# Autodesk Inventor assembly: 組合1
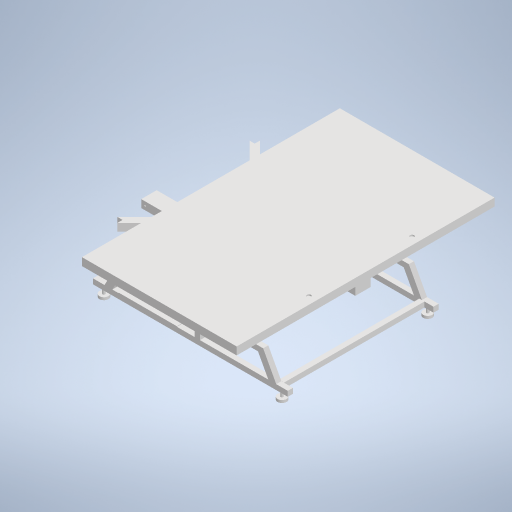
[picture p0: Inventor's stored thumbnail of the model, 512x512]
Saved by Autodesk Inventor 2024 (Build 280153000, 153)
## iProperties
Created: 2024-10-15
Part Number: 組合1
Document SubType Name: Assembly
Designer: jerry
Author: jerry
## Documents named in this file (21)
- C:\HeadTurner\HeadTurner\Linear Actuator\CAD Models\Inventor Model\組合1.iam
- C:\HeadTurner\HeadTurner\Linear Actuator\CAD Models\Inventor Model\Body Actuator.ipt
- C:\HeadTurner\HeadTurner\Linear Actuator\CAD Models\Inventor Model\DOF1.ipt
- C:\HeadTurner\HeadTurner\Linear Actuator\CAD Models\Inventor Model\DOF2.ipt
- C:\HeadTurner\HeadTurner\Linear Actuator\CAD Models\Inventor Model\DOF3.ipt
- C:\HeadTurner\HeadTurner\Linear Actuator\CAD Models\Inventor Model\DOF4.ipt
- C:\HeadTurner\HeadTurner\Linear Actuator\CAD Models\Inventor Model\DOF5.ipt
- C:\HeadTurner\HeadTurner\Linear Actuator\CAD Models\Inventor Model\DOF6.ipt
- C:\HeadTurner\HeadTurner\Linear Actuator\CAD Models\Inventor Model\DOF7.ipt
- C:\HeadTurner\HeadTurner\Linear Actuator\CAD Models\Inventor Model\DOF8.ipt
- C:\HeadTurner\HeadTurner\Linear Actuator\CAD Models\Inventor Model\DOF9.ipt
- C:\HeadTurner\HeadTurner\Linear Actuator\CAD Models\Inventor Model\DOF10.ipt
- C:\Users\jerry\OneDrive\Documents\Mattress.ipt
- C:\Users\jerry\OneDrive\Documents\Mattress2.ipt
- C:\Users\jerry\OneDrive\Documents\DOF11.ipt
- C:\Users\jerry\OneDrive\Documents\MotorPart1.ipt
- C:\Users\jerry\OneDrive\Documents\MotorPart2.ipt
- C:\Users\jerry\OneDrive\Documents\MotorPart3.ipt
- C:\Users\jerry\OneDrive\Documents\Cranker1.ipt
- C:\Users\jerry\OneDrive\Documents\MotorPart3_MIR.ipt
- C:\Users\jerry\OneDrive\Documents\Cranker1_MIR.ipt
## Components (22 placed, 20 different names)
1. Body Actuator:1 — 齊平:1, 齊平:3, 齊平:11
2. DOF1:1 — 齊平:1, 齊平:2
3. DOF2:1 — 齊平:2, 齊平:4, 齊平:6
4. DOF3:1 — 齊平:3
5. DOF4:1 — 齊平:4, 齊平:5
6. DOF5:1 — 齊平:5, 齊平:7, 齊平:8
7. DOF6:1 — 齊平:6, 齊平:13, 貼合:1, 貼合:2
8. DOF7:1 — 齊平:7, 齊平:10
9. DOF8:1 — 齊平:8, 齊平:9
10. DOF9:1 — 齊平:9
11. DOF10:1 — 齊平:10, 齊平:14, 貼合:3, 貼合:4
12. Mattress:1 — 齊平:11, 齊平:12
13. Mattress2:1 — 齊平:12
14. DOF11:1 — 齊平:13, 貼合:1, 貼合:2
15. MotorPart1:1 — 齊平:14, 貼合:3, 插入:1, 貼合:5
16. MotorPart1:2 — 貼合:4, 齊平:15, 齊平:16
17. MotorPart2:1 — 齊平:15
18. MotorPart2:2 — 插入:1
19. MotorPart3:1 — 齊平:16, 齊平:17
20. Cranker1:1 — 齊平:17
21. MotorPart3_MIR:1 — 貼合:5, 貼合:6
22. Cranker1_MIR:1 — 貼合:6
## Relationships (24: Flush 17, Mate 6, Insert 1)
- 齊平:1 [Flush]: Body Actuator:1 ↔ DOF1:1
- 齊平:2 [Flush]: DOF1:1 ↔ DOF2:1
- 齊平:3 [Flush]: Body Actuator:1 ↔ DOF3:1
- 齊平:4 [Flush]: DOF2:1 ↔ DOF4:1
- 齊平:5 [Flush]: DOF4:1 ↔ DOF5:1
- 齊平:6 [Flush]: DOF2:1 ↔ DOF6:1
- 齊平:7 [Flush]: DOF5:1 ↔ DOF7:1
- 齊平:8 [Flush]: DOF5:1 ↔ DOF8:1
- 齊平:9 [Flush]: DOF8:1 ↔ DOF9:1
- 齊平:10 [Flush]: DOF7:1 ↔ DOF10:1
- 齊平:11 [Flush]: Body Actuator:1 ↔ Mattress:1
- 齊平:12 [Flush]: Mattress:1 ↔ Mattress2:1
- 齊平:13 [Flush]: DOF6:1 ↔ DOF11:1
- 貼合:1 [Mate]: DOF6:1 ↔ DOF11:1
- 貼合:2 [Mate]: DOF6:1 ↔ DOF11:1
- 齊平:14 [Flush]: DOF10:1 ↔ MotorPart1:1
- 貼合:3 [Mate]: DOF10:1 ↔ MotorPart1:1
- 貼合:4 [Mate]: DOF10:1 ↔ MotorPart1:2
- 齊平:15 [Flush]: MotorPart1:2 ↔ MotorPart2:1
- 插入:1 [Insert]: MotorPart1:1 ↔ MotorPart2:2
- 齊平:16 [Flush]: MotorPart1:2 ↔ MotorPart3:1
- 齊平:17 [Flush]: MotorPart3:1 ↔ Cranker1:1
- 貼合:5 [Mate]: MotorPart1:1 ↔ MotorPart3_MIR:1
- 貼合:6 [Mate]: MotorPart3_MIR:1 ↔ Cranker1_MIR:1
